# Autodesk Inventor assembly: Molde_Completo
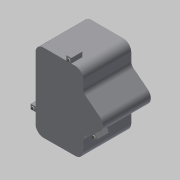
[picture p0: Inventor's stored thumbnail of the model, 180x180]
Saved by Autodesk Inventor 2019 (Build 230136000, 136)
## iProperties
Created: 2019-06-01
Part Number: Molde_Completo
Document SubType Name: Assembly
Designer: Emily Rojas
Author: Emily Rojas
## Documents named in this file (5)
- C:\Users\gusta\Documents\UPB\Diseño\Examen 1P\Ejercicio_2_Corregido\Molde_Completo.iam
- C:\Users\gusta\Documents\UPB\Diseño\Examen 1P\Ejercicio_2_Corregido\Molde_Cavidad.ipt
- C:\Users\gusta\Documents\UPB\Diseño\Examen 1P\Ejercicio_2_Corregido\Molde_Corazon.ipt
- C:\Users\gusta\Documents\UPB\Diseño\Examen 1P\Ejercicio_2_Corregido\AS 1110 - M5 x 40.ipt
- C:\Users\gusta\Documents\UPB\Diseño\Examen 1P\Ejercicio_2_Corregido\AS 1112 - M5(2).ipt
## Components (8 placed, 4 different names)
1. Molde_Cavidad:1 — Mate:1, Mate:2, Mate:3, Mate:10, Mate:11, Mate:12
2. Molde_Corazon:1 — Mate:1, Mate:2, Mate:3, Mate:4, Mate:5, Mate:6, Mate:7, Mate:8, Mate:9
3. AS 1110 - Metric M5 x 40:1 — Mate:7, Mate:11, Mate:14
4. AS 1112 (4) - Metric M5:1 — Mate:4, Mate:14
5. AS 1110 - Metric M5 x 40:2 — Mate:9, Mate:10, Mate:15
6. AS 1112 (4) - Metric M5:2 — Mate:5, Mate:15
7. AS 1110 - Metric M5 x 40:3 — Mate:8, Mate:12, Mate:13
8. AS 1112 (4) - Metric M5:3 — Mate:6, Mate:13
## Relationships (15: Mate 15)
- Mate:1: Molde_Cavidad:1 ↔ Molde_Corazon:1
- Mate:2: Molde_Cavidad:1 ↔ Molde_Corazon:1
- Mate:3: Molde_Cavidad:1 ↔ Molde_Corazon:1
- Mate:4: Molde_Corazon:1 ↔ AS 1112 (4) - Metric M5:1
- Mate:5: Molde_Corazon:1 ↔ AS 1112 (4) - Metric M5:2
- Mate:6: Molde_Corazon:1 ↔ AS 1112 (4) - Metric M5:3
- Mate:7: Molde_Corazon:1 ↔ AS 1110 - Metric M5 x 40:1
- Mate:8: Molde_Corazon:1 ↔ AS 1110 - Metric M5 x 40:3
- Mate:9: Molde_Corazon:1 ↔ AS 1110 - Metric M5 x 40:2
- Mate:10: Molde_Cavidad:1 ↔ AS 1110 - Metric M5 x 40:2
- Mate:11: Molde_Cavidad:1 ↔ AS 1110 - Metric M5 x 40:1
- Mate:12: Molde_Cavidad:1 ↔ AS 1110 - Metric M5 x 40:3
- Mate:13: AS 1110 - Metric M5 x 40:3 ↔ AS 1112 (4) - Metric M5:3
- Mate:14: AS 1110 - Metric M5 x 40:1 ↔ AS 1112 (4) - Metric M5:1
- Mate:15: AS 1110 - Metric M5 x 40:2 ↔ AS 1112 (4) - Metric M5:2
